# Autodesk Inventor assembly: test_hand
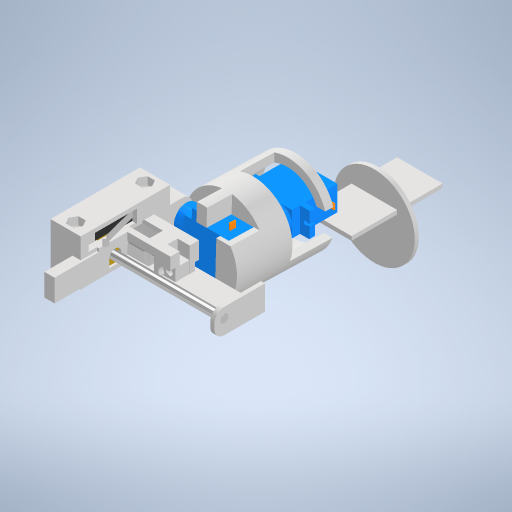
[picture p0: Inventor's stored thumbnail of the model, 512x512]
Saved by Autodesk Inventor 2024.1 (Build 281209000, 209)
## iProperties
Created: 2025-01-23
Part Number: test_hand
Document SubType Name: Assembly
Designer: hibik
Author: hibik
## Documents named in this file (9)
- C:\Users\hibik\Documents\Robomech\RESCUE\ORCA\hard\arm\test_hand.iam
- C:\Users\hibik\Documents\Robomech\RESCUE\ORCA\hard\std_parts\motor_M4_55.ipt
- C:\Users\hibik\Documents\Robomech\RESCUE\ORCA\hard\std_parts\limit_switch.ipt
- C:\Users\hibik\Documents\Robomech\RESCUE\ORCA\hard\std_parts\Miusei_ms18.ipt
- C:\Users\hibik\Documents\Robomech\RESCUE\ORCA\hard\arm\hand_motor_setter_base.ipt
- C:\Users\hibik\Documents\Robomech\RESCUE\ORCA\hard\arm\hand_motor_setter_cover_under.ipt
- C:\Users\hibik\Documents\Robomech\RESCUE\ORCA\hard\arm\wrist_wrist.ipt
- C:\Users\hibik\Documents\Robomech\RESCUE\ORCA\hard\arm\wrist_geard_hone.ipt
- C:\Users\hibik\Documents\Robomech\RESCUE\ORCA\hard\arm\arm_2.ipt
## Components (9 placed, 8 different names)
1. limit_switch:1 — メイト:1, メイト:2, メイト:3
2. Miusei_ms18:1 — 挿入:4, メイト:4, メイト:5, メイト:6
3. motor_M4_55:1 — 挿入:1, 角度:1
4. hand_motor_setter_base:1 — 挿入:1, 角度:1, メイト:1, メイト:2, メイト:3, 挿入:2, 挿入:3, 挿入:4
5. hand_motor_setter_cover_under:1 — 挿入:2, 挿入:3
6. wrist_wrist:1 — メイト:4, メイト:5, メイト:6
7. Miusei_ms18:2
8. wrist_geard_hone:2
9. arm_2:1
## Relationships (11: Mate 6, Insert 4, Angle 1)
- 挿入:1 [Insert] (0.1 mm): motor_M4_55:1 ↔ hand_motor_setter_base:1
- 角度:1 [Angle] (0 deg): motor_M4_55:1 ↔ hand_motor_setter_base:1
- メイト:1 [Mate] (0.1 mm): limit_switch:1 ↔ hand_motor_setter_base:1
- メイト:2 [Mate] (0.1 mm): limit_switch:1 ↔ hand_motor_setter_base:1
- メイト:3 [Mate] (0.1 mm): limit_switch:1 ↔ hand_motor_setter_base:1
- 挿入:2 [Insert]: hand_motor_setter_base:1 ↔ hand_motor_setter_cover_under:1
- 挿入:3 [Insert]: hand_motor_setter_base:1 ↔ hand_motor_setter_cover_under:1
- 挿入:4 [Insert] (1 mm): Miusei_ms18:1 ↔ hand_motor_setter_base:1
- メイト:4 [Mate]: Miusei_ms18:1 ↔ wrist_wrist:1
- メイト:5 [Mate]: Miusei_ms18:1 ↔ wrist_wrist:1
- メイト:6 [Mate] (0.1 mm): Miusei_ms18:1 ↔ wrist_wrist:1
